(part 1 of 2)
# Autodesk Inventor assembly: testframe
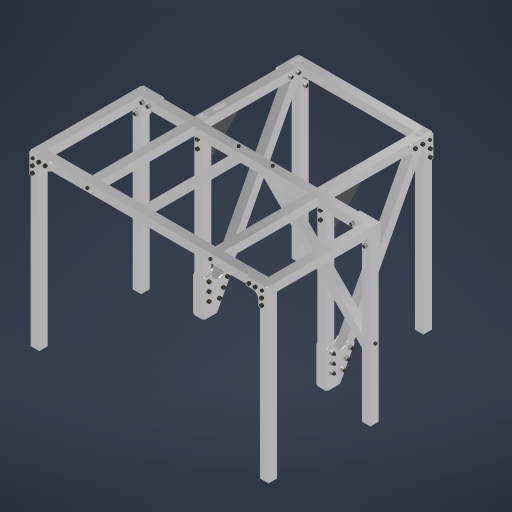
[picture p0: Inventor's stored thumbnail of the model, 512x512]
Saved by Autodesk Inventor 2024.2 (Build 282272000, 272)
## iProperties
Created: 2024-07-23
Part Number: testframe
Document SubType Name: Assembly
Designer: bryan
Mass: 9363.54 g
Surface Area: 20423.1 cm^2
Volume: 3333.5 cm^3
Density: 2.80893 g/cm^3
Author: bryan
## Documents named in this file (28)
- C:\Users\bobsb\OneDrive\Documents\GitHub\1622-2024-Summer-CAD-A-Thon\Structure\STRU_000_StructureAssembly.iam
- C:\Users\bobsb\OneDrive\Documents\GitHub\1622-2024-Summer-CAD-A-Thon\Structure\STRU_001_BilletBlock.ipt
- C:\Users\bobsb\OneDrive\Documents\GitHub\1622-2024-Summer-CAD-A-Thon\Structure\STRU_002_BilletPole_20.56in_Angled.ipt
- C:\Users\bobsb\OneDrive\Documents\GitHub\1622-2024-Summer-CAD-A-Thon\Structure\STRU_003_BilletPole_28in_Angled.ipt
- C:\Users\bobsb\OneDrive\Documents\GitHub\1622-2024-Summer-CAD-A-Thon\Structure\STRU_004_DoubleBillet_90_2.25in.ipt
- C:\Users\bobsb\OneDrive\Documents\GitHub\1622-2024-Summer-CAD-A-Thon\Structure\STRU_007_BilletPole_11in.ipt
- C:\Users\bobsb\OneDrive\Documents\GitHub\1622-2024-Summer-CAD-A-Thon\Structure\STRU_003_BilletPole_28in_Angled_Unique.ipt
- C:\Users\bobsb\OneDrive\Documents\GitHub\1622-2024-Summer-CAD-A-Thon\COTS Library\Fasteners\Bolts\Socket-Head\10-32\COTS_90044A120_Black-Oxide Alloy Steel Socket Head Screw.ipt
- C:\Users\bobsb\OneDrive\Documents\GitHub\1622-2024-Summer-CAD-A-Thon\COTS Library\Fasteners\Bolts\Socket-Head\0.25-20\COTS_90044A123_Black-Oxide Alloy Steel Socket Head Screw.ipt
- C:\Users\bobsb\OneDrive\Documents\GitHub\1622-2024-Summer-CAD-A-Thon\COTS Library\Fasteners\Nuts\COTS_95615A120_Medium-Strength Steel Nylon-Insert Locknut.ipt
- C:\Users\bobsb\OneDrive\Documents\GitHub\1622-2024-Summer-CAD-A-Thon\Structure\STRU_009_FrameBracket_90.ipt
- C:\Users\bobsb\OneDrive\Documents\GitHub\1622-2024-Summer-CAD-A-Thon\Structure\STRU_006_BilletPole_SwerveOffset.ipt
- C:\Users\bobsb\OneDrive\Documents\GitHub\1622-2024-Summer-CAD-A-Thon\Structure\STRU_010_BilletCrossbar_Angled.ipt
- C:\Users\bobsb\OneDrive\Documents\GitHub\1622-2024-Summer-CAD-A-Thon\Structure\STRU_011_BilletWedge.ipt
- C:\Users\bobsb\OneDrive\Documents\GitHub\1622-2024-Summer-CAD-A-Thon\COTS Library\Fasteners\Bolts\Socket-Head\10-32\COTS_90044A119_Black-Oxide Alloy Steel Socket Head Screw.ipt
- C:\Users\bobsb\OneDrive\Documents\GitHub\1622-2024-Summer-CAD-A-Thon\Structure\STRU_012_BilletPoleMiddle.ipt
- C:\Users\bobsb\OneDrive\Documents\GitHub\1622-2024-Summer-CAD-A-Thon\Structure\STRU_013_BilletCrossbar2_Angled.ipt
- C:\Users\bobsb\OneDrive\Documents\GitHub\1622-2024-Summer-CAD-A-Thon\Structure\STRU_012_BilletPoleMiddle_Unique.ipt
- C:\Users\bobsb\OneDrive\Documents\GitHub\1622-2024-Summer-CAD-A-Thon\Structure\STRU_014_BilletPole_9in_Angled.ipt
- C:\Users\bobsb\OneDrive\Documents\GitHub\1622-2024-Summer-CAD-A-Thon\Structure\STRU_015_BilletPole_9in.ipt
- C:\Users\bobsb\OneDrive\Documents\GitHub\1622-2024-Summer-CAD-A-Thon\Structure\STRU_016_FrameBracket2_90.ipt
- C:\Users\bobsb\OneDrive\Documents\GitHub\1622-2024-Summer-CAD-A-Thon\Structure\STRU_017_AngleBracket_90_Plastic.ipt
- C:\Users\bobsb\OneDrive\Documents\GitHub\1622-2024-Summer-CAD-A-Thon\Structure\STRU_018_AngleBracket_62.ipt
- C:\Users\bobsb\OneDrive\Documents\GitHub\1622-2024-Summer-CAD-A-Thon\COTS Library\Fasteners\Bolts\Socket-Head\0.25-20\COTS_91251A539_Black-Oxide Alloy Steel Socket Head Screw (1).ipt
- C:\Users\bobsb\OneDrive\Documents\GitHub\1622-2024-Summer-CAD-A-Thon\COTS Library\Fasteners\Bolts\Socket-Head\0.25-20\COTS_90044A124_Black-Oxide Alloy Steel Socket Head Screw.ipt
- C:\Users\bobsb\OneDrive\Documents\GitHub\1622-2024-Summer-CAD-A-Thon\COTS Library\Fasteners\Nuts\COTS_95462A029_Medium-Strength Steel Hex Nut (2).ipt
- C:\Users\bobsb\OneDrive\Documents\GitHub\1622-2024-Summer-CAD-A-Thon\Structure\STRU_019_RubberWasher.ipt
- C:\Users\bobsb\OneDrive\Documents\GitHub\1622-2024-Summer-CAD-A-Thon\Structure\STRU_000_StructureAssembly\AIP\FEA\err5tqxb5.fres
## Components (169 placed, 26 different names)
1. STRU_001_BilletBlock:2 — Mate:16, Mate:17, Flush:2
2. STRU_002_BilletPole_20.56in_Angled:1 — Mate:1, Mate:4, Mate:5, Mate:41, Mate:53, Mate:54, Flush:10, Mate:91, Mate:92, Mate:127, Mate:147, Mate:148, Mate:209, Mate:211, Mate:212, Mate:213, Mate:411
3. STRU_004_DoubleBillet_90_2.25in:1 — Mate:1, Mate:4, Mate:5, Mate:34, Mate:56, Mate:58, Mate:125, Mate:126
4. STRU_002_BilletPole_20.56in_Angled:2 — Mate:13, Mate:14, Mate:15, Mate:16, Mate:17, Flush:2, Mate:40, Mate:85, Mate:86, Mate:123, Mate:124, Mate:145, Mate:146, Mate:200, Mate:201, Mate:218, Mate:219, Mate:415
5. STRU_004_DoubleBillet_90_2.25in:2 — Mate:13, Mate:14, Mate:15, Mate:36, Mate:57, Mate:100, Mate:121, Mate:122
6. STRU_001_BilletBlock:3 — Mate:185, Mate:186, Flush:26
7. STRU_001_BilletBlock:4 — Mate:180, Mate:181, Flush:25
8. STRU_003_BilletPole_28in_Angled:2 — Mate:47, Flush:8, Flush:9, Mate:55, Mate:74, Mate:79, Mate:80, Mate:87, Mate:88, Mate:97, Mate:118, Mate:130, Mate:140, Mate:153, Mate:154, Mate:155, Mate:156, Mate:157, Mate:158, Mate:161, Mate:163, Mate:168, Mate:173, Flush:24, Mate:176, Mate:178, Mate:182
9. STRU_004_DoubleBillet_90_2.25in:3 — Mate:35, Mate:128, Mate:129, Mate:184
10. STRU_004_DoubleBillet_90_2.25in:4 — Mate:37, Mate:119, Mate:120, Mate:179
11. STRU_001_BilletBlock:5 — Mate:34, Mate:41, Mate:50, Mate:51
12. STRU_001_BilletBlock:6 — Mate:35, Mate:48, Mate:49
13. STRU_001_BilletBlock:7 — Mate:37, Mate:45, Mate:46
14. STRU_001_BilletBlock:8 — Mate:36, Mate:40, Mate:42, Mate:43
15. STRU_007_BilletPole_11in:1 — Mate:48, Mate:49, Flush:9, Mate:50, Mate:51, Mate:55, Mate:59
16. STRU_007_BilletPole_11in:2 — Mate:42, Mate:43, Mate:45, Mate:46, Mate:47, Flush:8, Mate:124
17. STRU_001_BilletBlock:9 — Mate:53, Mate:54, Flush:10
18. STRU_003_BilletPole_28in_Angled_Unique:1 — Mate:56, Mate:57, Mate:58, Mate:59, Mate:83, Mate:84, Mate:93, Mate:94, Mate:98, Mate:149, Mate:150, Mate:151, Mate:152, Mate:159, Mate:160, Mate:164, Mate:165, Flush:27, Mate:203, Mate:205, Mate:206, Mate:208, Mate:214, Mate:215, Mate:216, Mate:217, Flush:28, Mate:221, Flush:29, Mate:223, Mate:261, Mate:262, Mate:408, Mate:412
19. STRU_001_BilletBlock:10 — Mate:74, Mate:157, Mate:172
20. COTS_90044A120_Black-Oxide Alloy Steel Socket Head Screw:1 — Mate:142, Mate:193
21. COTS_90044A123_Black-Oxide Alloy Steel Socket Head Screw:2 — Mate:80, Mate:102, Mate:141, Flush:21
22. COTS_90044A123_Black-Oxide Alloy Steel Socket Head Screw:3 — Mate:103, Flush:22, Flush:23, Mate:191
23. COTS_90044A123_Black-Oxide Alloy Steel Socket Head Screw:4 — Mate:79, Mate:101, Flush:21, Flush:22
24. COTS_90044A123_Black-Oxide Alloy Steel Socket Head Screw:5 — Mate:104, Flush:23, Mate:192
25. COTS_90044A123_Black-Oxide Alloy Steel Socket Head Screw:6 — Mate:84, Mate:108, Flush:12
26. COTS_90044A123_Black-Oxide Alloy Steel Socket Head Screw:7 — Mate:85, Mate:106, Mate:134, Flush:12, Flush:13, Flush:14
27. COTS_90044A123_Black-Oxide Alloy Steel Socket Head Screw:8 — Mate:83, Mate:107, Flush:13
28. COTS_90044A123_Black-Oxide Alloy Steel Socket Head Screw:9 — Mate:86, Mate:105, Flush:14
29. COTS_90044A123_Black-Oxide Alloy Steel Socket Head Screw:10 — Mate:112, Flush:18, Mate:188
30. COTS_90044A123_Black-Oxide Alloy Steel Socket Head Screw:11 — Mate:111, Mate:139, Flush:18, Flush:19, Flush:20, Mate:187
31. COTS_90044A123_Black-Oxide Alloy Steel Socket Head Screw:12 — Mate:88, Mate:110, Flush:20
32. COTS_90044A123_Black-Oxide Alloy Steel Socket Head Screw:13 — Mate:87, Mate:109, Flush:19
33. COTS_90044A123_Black-Oxide Alloy Steel Socket Head Screw:14 — Mate:93, Mate:115, Flush:16
34. COTS_90044A123_Black-Oxide Alloy Steel Socket Head Screw:15 — Mate:92, Mate:114, Flush:17
35. COTS_90044A123_Black-Oxide Alloy Steel Socket Head Screw:16 — Mate:91, Mate:113, Mate:136, Flush:15, Flush:17
36. COTS_90044A123_Black-Oxide Alloy Steel Socket Head Screw:17 — Mate:94, Mate:116, Flush:15, Flush:16
37. COTS_90044A120_Black-Oxide Alloy Steel Socket Head Screw:3 — Mate:140, Mate:158
38. COTS_90044A120_Black-Oxide Alloy Steel Socket Head Screw:5 — Mate:97, Mate:138
39. COTS_90044A120_Black-Oxide Alloy Steel Socket Head Screw:6 — Mate:100, Mate:135
40. COTS_90044A120_Black-Oxide Alloy Steel Socket Head Screw:7 — Mate:98, Mate:137
41. COTS_95615A120_Medium-Strength Steel Nylon-Insert Locknut:1 — Mate:102, Mate:154
42. COTS_95615A120_Medium-Strength Steel Nylon-Insert Locknut:2 — Mate:101, Mate:153
43. COTS_95615A120_Medium-Strength Steel Nylon-Insert Locknut:3 — Mate:103, Mate:194
44. COTS_95615A120_Medium-Strength Steel Nylon-Insert Locknut:4 — Mate:104, Mate:195
45. COTS_95615A120_Medium-Strength Steel Nylon-Insert Locknut:5 — Mate:107, Mate:152
46. COTS_95615A120_Medium-Strength Steel Nylon-Insert Locknut:6 — Mate:108, Mate:151
47. COTS_95615A120_Medium-Strength Steel Nylon-Insert Locknut:7 — Mate:105, Mate:145
48. COTS_95615A120_Medium-Strength Steel Nylon-Insert Locknut:8 — Mate:106, Mate:146
49. COTS_95615A120_Medium-Strength Steel Nylon-Insert Locknut:9 — Mate:109, Mate:155
50. COTS_95615A120_Medium-Strength Steel Nylon-Insert Locknut:10 — Mate:110, Mate:156
51. COTS_95615A120_Medium-Strength Steel Nylon-Insert Locknut:11 — Mate:111, Mate:189
52. COTS_95615A120_Medium-Strength Steel Nylon-Insert Locknut:12 — Mate:112, Mate:190
53. COTS_95615A120_Medium-Strength Steel Nylon-Insert Locknut:13 — Mate:114, Mate:147
54. COTS_95615A120_Medium-Strength Steel Nylon-Insert Locknut:14 — Mate:113, Mate:148
55. COTS_95615A120_Medium-Strength Steel Nylon-Insert Locknut:15 — Mate:115, Mate:149
56. COTS_95615A120_Medium-Strength Steel Nylon-Insert Locknut:16 — Mate:116, Mate:150
57. STRU_009_FrameBracket_90:1 — Mate:118, Mate:119, Mate:120, Mate:141, Mate:142, Mate:177, Mate:191, Mate:192, Mate:193
58. STRU_009_FrameBracket_90:2 — Mate:125, Mate:126, Mate:127, Mate:136, Mate:137
59. STRU_009_FrameBracket_90:3 — Mate:121, Mate:122, Mate:123, Mate:134, Mate:135
60. STRU_009_FrameBracket_90:4 — Mate:128, Mate:129, Mate:130, Mate:138, Mate:139, Mate:183, Mate:187, Mate:188
61. STRU_001_BilletBlock:11 — Mate:159, Mate:165, Mate:171
62. STRU_001_BilletBlock:12 — Mate:160, Mate:164, Mate:174
63. STRU_001_BilletBlock:13 — Mate:161, Mate:162, Mate:163, Mate:175
64. COTS_90044A120_Black-Oxide Alloy Steel Socket Head Screw:10 — Mate:162, Mate:168
65. STRU_007_BilletPole_11in:3 — Mate:171, Mate:172, Mate:173, Flush:27
66. STRU_007_BilletPole_11in:4 — Mate:174, Mate:175, Flush:24, Mate:176
67. STRU_006_BilletPole_SwerveOffset:1 — Mate:177, Mate:178, Mate:179, Mate:180, Mate:181, Flush:25, Mate:194, Mate:195
68. STRU_006_BilletPole_SwerveOffset:2 — Mate:182, Mate:183, Mate:184, Mate:185, Mate:186, Flush:26, Mate:189, Mate:190
69. STRU_011_BilletWedge:1 — Mate:200, Mate:201, Mate:414
70. STRU_011_BilletWedge:3 — Mate:203, Mate:205, Mate:413
71. STRU_011_BilletWedge:4 — Mate:206, Mate:208, Mate:409
72. STRU_011_BilletWedge:5 — Mate:209, Mate:211, Mate:410
73. COTS_90044A119_Black-Oxide Alloy Steel Socket Head Screw:1 — Mate:212, Mate:213
74. COTS_90044A119_Black-Oxide Alloy Steel Socket Head Screw:2 — Mate:214, Mate:215
75. COTS_90044A119_Black-Oxide Alloy Steel Socket Head Screw:3 — Mate:216, Mate:217
76. COTS_90044A119_Black-Oxide Alloy Steel Socket Head Screw:4 — Mate:218, Mate:219
77. STRU_012_BilletPoleMiddle:6 — Flush:28, Mate:221, Mate:228, Mate:229, Flush:30, Flush:43, Mate:251, Mate:255, Flush:49, Mate:261, Mate:263, Mate:318, Mate:324, Mate:331, Mate:389, Mate:390, Mate:418, Mate:419
78. STRU_012_BilletPoleMiddle:5 — Flush:29, Mate:223, Mate:230, Mate:231, Flush:31, Flush:39, Mate:233, Mate:234, Mate:249, Mate:253, Flush:48, Mate:262, Mate:264, Mate:319, Mate:321, Mate:328, Mate:391, Mate:392, Mate:416, Mate:417
79. STRU_001_BilletBlock:14 — Mate:228, Mate:229, Flush:30
80. STRU_001_BilletBlock:15 — Mate:230, Mate:231, Flush:31
81. STRU_013_BilletCrossbar2_Angled:1 — Flush:39, Mate:233, Mate:234, Mate:252, Mate:273, Flush:56, Flush:57, Mate:287, Mate:322, Mate:323, Mate:327, Mate:329
82. STRU_013_BilletCrossbar2_Angled:3 — Flush:43, Mate:254, Mate:274, Flush:58, Mate:308, Mate:325, Mate:326, Mate:330, Mate:332
83. STRU_001_BilletBlock:16 — Mate:267, Mate:268, Flush:54
84. STRU_001_BilletBlock:17 — Mate:269, Mate:270, Flush:55
85. COTS_90044A120_Black-Oxide Alloy Steel Socket Head Screw:11 — Mate:249, Mate:264
86. COTS_90044A120_Black-Oxide Alloy Steel Socket Head Screw:12 — Mate:251, Mate:263
87. STRU_014_BilletPole_9in_Angled:1 — Mate:254, Mate:255, Flush:49, Mate:311, Mate:317, Mate:333, Mate:334, Mate:335, Mate:336
88. STRU_014_BilletPole_9in_Angled:2 — Mate:252, Mate:253, Flush:48, Mate:291, Mate:320, Mate:337, Mate:338, Mate:339, Mate:340
89. STRU_015_BilletPole_9in:1 — Mate:257, Mate:258, Mate:259, Mate:260, Flush:52, Flush:53, Flush:57
90. STRU_001_BilletBlock:18 — Mate:259, Mate:260, Flush:52, Mate:266, Mate:271, Mate:275
91. STRU_001_BilletBlock:19 — Mate:257, Mate:258, Flush:53, Mate:265, Mate:272, Mate:276
92. STRU_012_BilletPoleMiddle_Unique:1 — Mate:265, Mate:267, Mate:268, Flush:54, Mate:272, Mate:274, Flush:58, Mate:277, Mate:278, Mate:279, Mate:304, Mate:316
93. STRU_012_BilletPoleMiddle_Unique:2 — Mate:266, Mate:269, Mate:270, Flush:55, Mate:271, Mate:273, Flush:56, Mate:281, Mate:282, Mate:283, Mate:295, Mate:299
94. COTS_90044A120_Black-Oxide Alloy Steel Socket Head Screw:13 — Mate:275, Mate:284
95. COTS_90044A120_Black-Oxide Alloy Steel Socket Head Screw:14 — Mate:276, Mate:280
96. STRU_016_FrameBracket2_90:1 — Mate:277, Mate:278, Mate:279, Mate:280, Mate:302, Mate:303, Mate:306, Mate:307, Mate:310, Mate:312, Mate:314, Mate:315
97. STRU_016_FrameBracket2_90:2 — Mate:281, Mate:282, Mate:283, Mate:284, Mate:286, Mate:288, Mate:290, Mate:292, Mate:294, Mate:296, Mate:298, Mate:300
98. COTS_90044A123_Black-Oxide Alloy Steel Socket Head Screw:18 — Mate:286, Mate:288
99. COTS_95615A120_Medium-Strength Steel Nylon-Insert Locknut:17 — Mate:287
100. COTS_90044A123_Black-Oxide Alloy Steel Socket Head Screw:19 — Mate:290, Mate:292
101. COTS_95615A120_Medium-Strength Steel Nylon-Insert Locknut:18 — Mate:291
102. COTS_90044A123_Black-Oxide Alloy Steel Socket Head Screw:20 — Mate:294, Mate:296
103. COTS_95615A120_Medium-Strength Steel Nylon-Insert Locknut:19 — Mate:295
104. COTS_90044A123_Black-Oxide Alloy Steel Socket Head Screw:21 — Mate:298, Mate:300
105. COTS_95615A120_Medium-Strength Steel Nylon-Insert Locknut:20 — Mate:299
106. COTS_90044A123_Black-Oxide Alloy Steel Socket Head Screw:22 — Mate:302, Mate:303
107. COTS_95615A120_Medium-Strength Steel Nylon-Insert Locknut:21 — Mate:304
108. COTS_90044A123_Black-Oxide Alloy Steel Socket Head Screw:23 — Mate:306, Mate:307
109. COTS_95615A120_Medium-Strength Steel Nylon-Insert Locknut:22 — Mate:308
110. COTS_90044A123_Black-Oxide Alloy Steel Socket Head Screw:24 — Mate:310, Mate:312
111. COTS_95615A120_Medium-Strength Steel Nylon-Insert Locknut:23 — Mate:311
112. COTS_90044A123_Black-Oxide Alloy Steel Socket Head Screw:25 — Mate:314, Mate:315
113. COTS_95615A120_Medium-Strength Steel Nylon-Insert Locknut:24 — Mate:316
114. STRU_017_AngleBracket_90_Plastic:1 — Mate:317, Mate:318, Mate:453, Mate:454, Mate:458, Mate:462, Mate:463, Mate:467
115. STRU_017_AngleBracket_90_Plastic:2 — Mate:319, Mate:320, Mate:434, Mate:435, Mate:440, Mate:444, Mate:445, Mate:449
116. STRU_018_AngleBracket_62:1 — Mate:327, Mate:328, Mate:329, Mate:393, Mate:394, Mate:395, Mate:396, Mate:397, Mate:398, Mate:399, Mate:400, Mate:401, Mate:402, Mate:403, Mate:404
117. STRU_018_AngleBracket_62:2 — Mate:330, Mate:331, Mate:332, Mate:359, Mate:360, Mate:361, Mate:362, Mate:363, Mate:364, Mate:383, Mate:384, Mate:385, Mate:386, Mate:387, Mate:388
118. STRU_018_AngleBracket_62:3 — Mate:321, Mate:322, Mate:323, Mate:426, Mate:427, Mate:428, Mate:429, Mate:430, Mate:431
119. STRU_018_AngleBracket_62:4 — Mate:324, Mate:325, Mate:326, Mate:377, Mate:378, Mate:379, Mate:380, Mate:381, Mate:382
120. COTS_91251A539_Black-Oxide Alloy Steel Socket Head Screw (1):1 — Mate:337, Mate:340, Mate:439
121. COTS_91251A539_Black-Oxide Alloy Steel Socket Head Screw (1):2 — Mate:338, Mate:339, Mate:432, Mate:433
122. COTS_91251A539_Black-Oxide Alloy Steel Socket Head Screw (1):4 — Mate:333, Mate:334, Mate:457
123. COTS_91251A539_Black-Oxide Alloy Steel Socket Head Screw (1):5 — Mate:335, Mate:336, Mate:452
124. COTS_95615A120_Medium-Strength Steel Nylon-Insert Locknut:25 — Mate:373, Mate:385
125. COTS_95615A120_Medium-Strength Steel Nylon-Insert Locknut:26 — Mate:372, Mate:384
126. COTS_95615A120_Medium-Strength Steel Nylon-Insert Locknut:27 — Mate:371, Mate:383
127. COTS_95615A120_Medium-Strength Steel Nylon-Insert Locknut:28 — Mate:376, Mate:388
128. COTS_95615A120_Medium-Strength Steel Nylon-Insert Locknut:29 — Mate:375, Mate:387
129. COTS_95615A120_Medium-Strength Steel Nylon-Insert Locknut:30 — Mate:374, Mate:386
130. COTS_90044A123_Black-Oxide Alloy Steel Socket Head Screw:27 — Mate:390, Mate:419, Mate:461
131. COTS_90044A123_Black-Oxide Alloy Steel Socket Head Screw:28 — Mate:389, Mate:418, Mate:466
132. COTS_90044A123_Black-Oxide Alloy Steel Socket Head Screw:29 — Mate:392, Mate:417, Mate:448
133. COTS_90044A123_Black-Oxide Alloy Steel Socket Head Screw:30 — Mate:391, Mate:416, Mate:442, Mate:443
134. COTS_90044A124_Black-Oxide Alloy Steel Socket Head Screw:1 — Mate:359, Mate:371, Mate:382
135. COTS_90044A124_Black-Oxide Alloy Steel Socket Head Screw:2 — Mate:361, Mate:373, Mate:378
136. COTS_90044A124_Black-Oxide Alloy Steel Socket Head Screw:3 — Mate:360, Mate:372, Mate:381
137. COTS_90044A124_Black-Oxide Alloy Steel Socket Head Screw:4 — Mate:393, Mate:399, Mate:421
138. COTS_90044A124_Black-Oxide Alloy Steel Socket Head Screw:5 — Mate:394, Mate:401, Mate:422
139. COTS_90044A124_Black-Oxide Alloy Steel Socket Head Screw:6 — Mate:395, Mate:400, Mate:423
140. COTS_90044A124_Black-Oxide Alloy Steel Socket Head Screw:7 — Mate:362, Mate:374, Mate:379
141. COTS_90044A124_Black-Oxide Alloy Steel Socket Head Screw:8 — Mate:363, Mate:375, Mate:380
142. COTS_90044A124_Black-Oxide Alloy Steel Socket Head Screw:9 — Mate:364, Mate:376, Mate:377
143. COTS_90044A124_Black-Oxide Alloy Steel Socket Head Screw:10 — Mate:396, Mate:404, Mate:425
144. COTS_90044A124_Black-Oxide Alloy Steel Socket Head Screw:11 — Mate:397, Mate:403, Mate:424
145. COTS_90044A124_Black-Oxide Alloy Steel Socket Head Screw:12 — Mate:398, Mate:402, Mate:420
146. STRU_010_BilletCrossbar_Angled:2 — Mate:408, Mate:409, Mate:410, Mate:411
147. STRU_010_BilletCrossbar_Angled:3 — Mate:412, Mate:413, Mate:414, Mate:415
148. COTS_95615A120_Medium-Strength Steel Nylon-Insert Locknut:31 — Mate:423, Mate:430
149. COTS_95615A120_Medium-Strength Steel Nylon-Insert Locknut:32 — Mate:421, Mate:426
150. COTS_95615A120_Medium-Strength Steel Nylon-Insert Locknut:33 — Mate:425, Mate:429
151. COTS_95615A120_Medium-Strength Steel Nylon-Insert Locknut:34 — Mate:420, Mate:427
152. COTS_95615A120_Medium-Strength Steel Nylon-Insert Locknut:35 — Mate:422, Mate:431
153. COTS_95615A120_Medium-Strength Steel Nylon-Insert Locknut:36 — Mate:424, Mate:428
154. COTS_95462A029_Medium-Strength Steel Hex Nut (2):1 — Mate:432, Mate:436
155. STRU_019_RubberWasher:1 — Mate:433, Mate:434, Mate:435, Mate:436, Flush:59
156. COTS_95462A029_Medium-Strength Steel Hex Nut (2):2 — Mate:438, Mate:439
157. STRU_019_RubberWasher:2 — Mate:438, Flush:59, Mate:440
158. COTS_95462A029_Medium-Strength Steel Hex Nut (2):3 — Mate:442
159. STRU_019_RubberWasher:3 — Mate:443, Mate:444, Mate:445, Flush:60
160. COTS_95462A029_Medium-Strength Steel Hex Nut (2):4 — Mate:447, Mate:448
161. STRU_019_RubberWasher:4 — Mate:447, Mate:449, Flush:60
162. COTS_95462A029_Medium-Strength Steel Hex Nut (2):5 — Mate:452
163. STRU_019_RubberWasher:5 — Mate:453, Mate:454, Flush:61
164. COTS_95462A029_Medium-Strength Steel Hex Nut (2):6 — Mate:457
165. STRU_019_RubberWasher:6 — Mate:458, Flush:61
166. COTS_95462A029_Medium-Strength Steel Hex Nut (2):7 — Mate:461
167. STRU_019_RubberWasher:7 — Mate:462, Mate:463, Flush:62
168. COTS_95462A029_Medium-Strength Steel Hex Nut (2):8 — Mate:466
169. STRU_019_RubberWasher:8 — Mate:467, Flush:62
## Relationships (390: Mate 351, Flush 39)
- Mate:1: STRU_002_BilletPole_20.56in_Angled:1 ↔ STRU_004_DoubleBillet_90_2.25in:1
- Mate:4: STRU_002_BilletPole_20.56in_Angled:1 ↔ STRU_004_DoubleBillet_90_2.25in:1
- Mate:5: STRU_002_BilletPole_20.56in_Angled:1 ↔ STRU_004_DoubleBillet_90_2.25in:1
- Mate:13: STRU_002_BilletPole_20.56in_Angled:2 ↔ STRU_004_DoubleBillet_90_2.25in:2
- Mate:14: STRU_002_BilletPole_20.56in_Angled:2 ↔ STRU_004_DoubleBillet_90_2.25in:2
- Mate:15: STRU_002_BilletPole_20.56in_Angled:2 ↔ STRU_004_DoubleBillet_90_2.25in:2
- Mate:16: STRU_001_BilletBlock:2 ↔ STRU_002_BilletPole_20.56in_Angled:2
- Mate:17: STRU_001_BilletBlock:2 ↔ STRU_002_BilletPole_20.56in_Angled:2
- Flush:2: STRU_001_BilletBlock:2 ↔ STRU_002_BilletPole_20.56in_Angled:2
- [Mate]: STRU_003_BilletPole_28in_Angled:2 ↔ STRU_004_DoubleBillet_90_2.25in:3
- [Mate]: STRU_003_BilletPole_28in_Angled:2 ↔ STRU_004_DoubleBillet_90_2.25in:3
- [Mate]: STRU_003_BilletPole_28in_Angled:2 ↔ STRU_004_DoubleBillet_90_2.25in:3
- [Mate]: STRU_003_BilletPole_28in_Angled:2 ↔ STRU_004_DoubleBillet_90_2.25in:4
- [Mate]: STRU_003_BilletPole_28in_Angled:2 ↔ STRU_004_DoubleBillet_90_2.25in:4
- [Mate]: STRU_003_BilletPole_28in_Angled:2 ↔ STRU_004_DoubleBillet_90_2.25in:4
- Mate:34: STRU_004_DoubleBillet_90_2.25in:1 ↔ STRU_001_BilletBlock:5
- Mate:35: STRU_004_DoubleBillet_90_2.25in:3 ↔ STRU_001_BilletBlock:6
- Mate:36: STRU_004_DoubleBillet_90_2.25in:2 ↔ STRU_001_BilletBlock:8
- Mate:37: STRU_004_DoubleBillet_90_2.25in:4 ↔ STRU_001_BilletBlock:7
- Mate:40: STRU_002_BilletPole_20.56in_Angled:2 ↔ STRU_001_BilletBlock:8
- Mate:41: STRU_002_BilletPole_20.56in_Angled:1 ↔ STRU_001_BilletBlock:5
- Mate:42: STRU_001_BilletBlock:8 ↔ STRU_007_BilletPole_11in:2
- Mate:43: STRU_001_BilletBlock:8 ↔ STRU_007_BilletPole_11in:2
- Mate:45: STRU_001_BilletBlock:7 ↔ STRU_007_BilletPole_11in:2
- Mate:46: STRU_001_BilletBlock:7 ↔ STRU_007_BilletPole_11in:2
- Mate:47: STRU_003_BilletPole_28in_Angled:2 ↔ STRU_007_BilletPole_11in:2
- Flush:8: STRU_003_BilletPole_28in_Angled:2 ↔ STRU_007_BilletPole_11in:2
- Mate:48: STRU_001_BilletBlock:6 ↔ STRU_007_BilletPole_11in:1
- Mate:49: STRU_001_BilletBlock:6 ↔ STRU_007_BilletPole_11in:1
- Flush:9: STRU_003_BilletPole_28in_Angled:2 ↔ STRU_007_BilletPole_11in:1
- Mate:50: STRU_001_BilletBlock:5 ↔ STRU_007_BilletPole_11in:1
- Mate:51: STRU_001_BilletBlock:5 ↔ STRU_007_BilletPole_11in:1
- Mate:53: STRU_002_BilletPole_20.56in_Angled:1 ↔ STRU_001_BilletBlock:9
- Mate:54: STRU_002_BilletPole_20.56in_Angled:1 ↔ STRU_001_BilletBlock:9
- Flush:10: STRU_002_BilletPole_20.56in_Angled:1 ↔ STRU_001_BilletBlock:9
- Mate:55: STRU_003_BilletPole_28in_Angled:2 ↔ STRU_007_BilletPole_11in:1
- Mate:56: STRU_004_DoubleBillet_90_2.25in:1 ↔ STRU_003_BilletPole_28in_Angled_Unique:1
- Mate:57: STRU_004_DoubleBillet_90_2.25in:2 ↔ STRU_003_BilletPole_28in_Angled_Unique:1
- Mate:58: STRU_004_DoubleBillet_90_2.25in:1 ↔ STRU_003_BilletPole_28in_Angled_Unique:1
- Mate:59: STRU_007_BilletPole_11in:1 ↔ STRU_003_BilletPole_28in_Angled_Unique:1
- Mate:74: STRU_003_BilletPole_28in_Angled:2 ↔ STRU_001_BilletBlock:10
- Mate:79: STRU_003_BilletPole_28in_Angled:2 ↔ COTS_90044A123_Black-Oxide Alloy Steel Socket Head Screw:4
- Mate:80: STRU_003_BilletPole_28in_Angled:2 ↔ COTS_90044A123_Black-Oxide Alloy Steel Socket Head Screw:2
- Mate:83: STRU_003_BilletPole_28in_Angled_Unique:1 ↔ COTS_90044A123_Black-Oxide Alloy Steel Socket Head Screw:8
- Mate:84: STRU_003_BilletPole_28in_Angled_Unique:1 ↔ COTS_90044A123_Black-Oxide Alloy Steel Socket Head Screw:6
- Mate:85: STRU_002_BilletPole_20.56in_Angled:2 ↔ COTS_90044A123_Black-Oxide Alloy Steel Socket Head Screw:7
- Mate:86: STRU_002_BilletPole_20.56in_Angled:2 ↔ COTS_90044A123_Black-Oxide Alloy Steel Socket Head Screw:9
- Mate:87: STRU_003_BilletPole_28in_Angled:2 ↔ COTS_90044A123_Black-Oxide Alloy Steel Socket Head Screw:13
- Mate:88: STRU_003_BilletPole_28in_Angled:2 ↔ COTS_90044A123_Black-Oxide Alloy Steel Socket Head Screw:12
- Mate:91: STRU_002_BilletPole_20.56in_Angled:1 ↔ COTS_90044A123_Black-Oxide Alloy Steel Socket Head Screw:16
- Mate:92: STRU_002_BilletPole_20.56in_Angled:1 ↔ COTS_90044A123_Black-Oxide Alloy Steel Socket Head Screw:15
- Mate:93: STRU_003_BilletPole_28in_Angled_Unique:1 ↔ COTS_90044A123_Black-Oxide Alloy Steel Socket Head Screw:14
- Mate:94: STRU_003_BilletPole_28in_Angled_Unique:1 ↔ COTS_90044A123_Black-Oxide Alloy Steel Socket Head Screw:17
- Mate:97: STRU_003_BilletPole_28in_Angled:2 ↔ COTS_90044A120_Black-Oxide Alloy Steel Socket Head Screw:5
- Mate:98: STRU_003_BilletPole_28in_Angled_Unique:1 ↔ COTS_90044A120_Black-Oxide Alloy Steel Socket Head Screw:7
- Mate:100: STRU_004_DoubleBillet_90_2.25in:2 ↔ COTS_90044A120_Black-Oxide Alloy Steel Socket Head Screw:6
- Mate:101: COTS_90044A123_Black-Oxide Alloy Steel Socket Head Screw:4 ↔ COTS_95615A120_Medium-Strength Steel Nylon-Insert Locknut:2
- Mate:102: COTS_90044A123_Black-Oxide Alloy Steel Socket Head Screw:2 ↔ COTS_95615A120_Medium-Strength Steel Nylon-Insert Locknut:1
- Mate:103: COTS_90044A123_Black-Oxide Alloy Steel Socket Head Screw:3 ↔ COTS_95615A120_Medium-Strength Steel Nylon-Insert Locknut:3
- Mate:104: COTS_90044A123_Black-Oxide Alloy Steel Socket Head Screw:5 ↔ COTS_95615A120_Medium-Strength Steel Nylon-Insert Locknut:4
- Mate:105: COTS_90044A123_Black-Oxide Alloy Steel Socket Head Screw:9 ↔ COTS_95615A120_Medium-Strength Steel Nylon-Insert Locknut:7
- Mate:106: COTS_90044A123_Black-Oxide Alloy Steel Socket Head Screw:7 ↔ COTS_95615A120_Medium-Strength Steel Nylon-Insert Locknut:8
- Mate:107: COTS_90044A123_Black-Oxide Alloy Steel Socket Head Screw:8 ↔ COTS_95615A120_Medium-Strength Steel Nylon-Insert Locknut:5
- Mate:108: COTS_90044A123_Black-Oxide Alloy Steel Socket Head Screw:6 ↔ COTS_95615A120_Medium-Strength Steel Nylon-Insert Locknut:6
- Mate:109: COTS_90044A123_Black-Oxide Alloy Steel Socket Head Screw:13 ↔ COTS_95615A120_Medium-Strength Steel Nylon-Insert Locknut:9
- Mate:110: COTS_90044A123_Black-Oxide Alloy Steel Socket Head Screw:12 ↔ COTS_95615A120_Medium-Strength Steel Nylon-Insert Locknut:10
- Mate:111: COTS_90044A123_Black-Oxide Alloy Steel Socket Head Screw:11 ↔ COTS_95615A120_Medium-Strength Steel Nylon-Insert Locknut:11
- Mate:112: COTS_90044A123_Black-Oxide Alloy Steel Socket Head Screw:10 ↔ COTS_95615A120_Medium-Strength Steel Nylon-Insert Locknut:12
- Mate:113: COTS_90044A123_Black-Oxide Alloy Steel Socket Head Screw:16 ↔ COTS_95615A120_Medium-Strength Steel Nylon-Insert Locknut:14
- Mate:114: COTS_90044A123_Black-Oxide Alloy Steel Socket Head Screw:15 ↔ COTS_95615A120_Medium-Strength Steel Nylon-Insert Locknut:13
- Mate:115: COTS_90044A123_Black-Oxide Alloy Steel Socket Head Screw:14 ↔ COTS_95615A120_Medium-Strength Steel Nylon-Insert Locknut:15
- Mate:116: COTS_90044A123_Black-Oxide Alloy Steel Socket Head Screw:17 ↔ COTS_95615A120_Medium-Strength Steel Nylon-Insert Locknut:16
- Mate:118: STRU_003_BilletPole_28in_Angled:2 ↔ STRU_009_FrameBracket_90:1
- Mate:119: STRU_004_DoubleBillet_90_2.25in:4 ↔ STRU_009_FrameBracket_90:1
- Mate:120: STRU_004_DoubleBillet_90_2.25in:4 ↔ STRU_009_FrameBracket_90:1
- Mate:121: STRU_004_DoubleBillet_90_2.25in:2 ↔ STRU_009_FrameBracket_90:3
- Mate:122: STRU_004_DoubleBillet_90_2.25in:2 ↔ STRU_009_FrameBracket_90:3
- Mate:123: STRU_002_BilletPole_20.56in_Angled:2 ↔ STRU_009_FrameBracket_90:3
- Mate:124: STRU_002_BilletPole_20.56in_Angled:2 ↔ STRU_007_BilletPole_11in:2
- Mate:125: STRU_004_DoubleBillet_90_2.25in:1 ↔ STRU_009_FrameBracket_90:2
- Mate:126: STRU_004_DoubleBillet_90_2.25in:1 ↔ STRU_009_FrameBracket_90:2
- Mate:127: STRU_002_BilletPole_20.56in_Angled:1 ↔ STRU_009_FrameBracket_90:2
- Mate:128: STRU_004_DoubleBillet_90_2.25in:3 ↔ STRU_009_FrameBracket_90:4
- Mate:129: STRU_004_DoubleBillet_90_2.25in:3 ↔ STRU_009_FrameBracket_90:4
- Mate:130: STRU_003_BilletPole_28in_Angled:2 ↔ STRU_009_FrameBracket_90:4
- Mate:134: COTS_90044A123_Black-Oxide Alloy Steel Socket Head Screw:7 ↔ STRU_009_FrameBracket_90:3
- Flush:12: COTS_90044A123_Black-Oxide Alloy Steel Socket Head Screw:6 ↔ COTS_90044A123_Black-Oxide Alloy Steel Socket Head Screw:7
- Mate:135: COTS_90044A120_Black-Oxide Alloy Steel Socket Head Screw:6 ↔ STRU_009_FrameBracket_90:3
- Flush:13: COTS_90044A123_Black-Oxide Alloy Steel Socket Head Screw:7 ↔ COTS_90044A123_Black-Oxide Alloy Steel Socket Head Screw:8
- Flush:14: COTS_90044A123_Black-Oxide Alloy Steel Socket Head Screw:7 ↔ COTS_90044A123_Black-Oxide Alloy Steel Socket Head Screw:9
- Mate:136: COTS_90044A123_Black-Oxide Alloy Steel Socket Head Screw:16 ↔ STRU_009_FrameBracket_90:2
- Mate:137: COTS_90044A120_Black-Oxide Alloy Steel Socket Head Screw:7 ↔ STRU_009_FrameBracket_90:2
- Flush:15: COTS_90044A123_Black-Oxide Alloy Steel Socket Head Screw:16 ↔ COTS_90044A123_Black-Oxide Alloy Steel Socket Head Screw:17
- Flush:16: COTS_90044A123_Black-Oxide Alloy Steel Socket Head Screw:14 ↔ COTS_90044A123_Black-Oxide Alloy Steel Socket Head Screw:17
- Flush:17: COTS_90044A123_Black-Oxide Alloy Steel Socket Head Screw:15 ↔ COTS_90044A123_Black-Oxide Alloy Steel Socket Head Screw:16
- Mate:138: COTS_90044A120_Black-Oxide Alloy Steel Socket Head Screw:5 ↔ STRU_009_FrameBracket_90:4
- Mate:139: COTS_90044A123_Black-Oxide Alloy Steel Socket Head Screw:11 ↔ STRU_009_FrameBracket_90:4
- Flush:18: COTS_90044A123_Black-Oxide Alloy Steel Socket Head Screw:10 ↔ COTS_90044A123_Black-Oxide Alloy Steel Socket Head Screw:11
- Flush:19: COTS_90044A123_Black-Oxide Alloy Steel Socket Head Screw:11 ↔ COTS_90044A123_Black-Oxide Alloy Steel Socket Head Screw:13
- Flush:20: COTS_90044A123_Black-Oxide Alloy Steel Socket Head Screw:11 ↔ COTS_90044A123_Black-Oxide Alloy Steel Socket Head Screw:12
- Mate:140: STRU_003_BilletPole_28in_Angled:2 ↔ COTS_90044A120_Black-Oxide Alloy Steel Socket Head Screw:3
- Mate:141: COTS_90044A123_Black-Oxide Alloy Steel Socket Head Screw:2 ↔ STRU_009_FrameBracket_90:1
- Mate:142: COTS_90044A120_Black-Oxide Alloy Steel Socket Head Screw:1 ↔ STRU_009_FrameBracket_90:1
- Flush:21: COTS_90044A123_Black-Oxide Alloy Steel Socket Head Screw:2 ↔ COTS_90044A123_Black-Oxide Alloy Steel Socket Head Screw:4
- Flush:22: COTS_90044A123_Black-Oxide Alloy Steel Socket Head Screw:3 ↔ COTS_90044A123_Black-Oxide Alloy Steel Socket Head Screw:4
- Flush:23: COTS_90044A123_Black-Oxide Alloy Steel Socket Head Screw:3 ↔ COTS_90044A123_Black-Oxide Alloy Steel Socket Head Screw:5
- Mate:145: STRU_002_BilletPole_20.56in_Angled:2 ↔ COTS_95615A120_Medium-Strength Steel Nylon-Insert Locknut:7
- Mate:146: STRU_002_BilletPole_20.56in_Angled:2 ↔ COTS_95615A120_Medium-Strength Steel Nylon-Insert Locknut:8
- Mate:147: STRU_002_BilletPole_20.56in_Angled:1 ↔ COTS_95615A120_Medium-Strength Steel Nylon-Insert Locknut:13
- Mate:148: STRU_002_BilletPole_20.56in_Angled:1 ↔ COTS_95615A120_Medium-Strength Steel Nylon-Insert Locknut:14
- Mate:149: STRU_003_BilletPole_28in_Angled_Unique:1 ↔ COTS_95615A120_Medium-Strength Steel Nylon-Insert Locknut:15
- Mate:150: STRU_003_BilletPole_28in_Angled_Unique:1 ↔ COTS_95615A120_Medium-Strength Steel Nylon-Insert Locknut:16
- Mate:151: STRU_003_BilletPole_28in_Angled_Unique:1 ↔ COTS_95615A120_Medium-Strength Steel Nylon-Insert Locknut:6
- Mate:152: STRU_003_BilletPole_28in_Angled_Unique:1 ↔ COTS_95615A120_Medium-Strength Steel Nylon-Insert Locknut:5
- Mate:153: STRU_003_BilletPole_28in_Angled:2 ↔ COTS_95615A120_Medium-Strength Steel Nylon-Insert Locknut:2
- Mate:154: STRU_003_BilletPole_28in_Angled:2 ↔ COTS_95615A120_Medium-Strength Steel Nylon-Insert Locknut:1
- Mate:155: STRU_003_BilletPole_28in_Angled:2 ↔ COTS_95615A120_Medium-Strength Steel Nylon-Insert Locknut:9
- Mate:156: STRU_003_BilletPole_28in_Angled:2 ↔ COTS_95615A120_Medium-Strength Steel Nylon-Insert Locknut:10
- Mate:157: STRU_003_BilletPole_28in_Angled:2 ↔ STRU_001_BilletBlock:10
- Mate:158: STRU_003_BilletPole_28in_Angled:2 ↔ COTS_90044A120_Black-Oxide Alloy Steel Socket Head Screw:3
- Mate:159: STRU_003_BilletPole_28in_Angled_Unique:1 ↔ STRU_001_BilletBlock:11
- Mate:160: STRU_003_BilletPole_28in_Angled_Unique:1 ↔ STRU_001_BilletBlock:12
- Mate:161: STRU_003_BilletPole_28in_Angled:2 ↔ STRU_001_BilletBlock:13
- Mate:162: STRU_001_BilletBlock:13 ↔ COTS_90044A120_Black-Oxide Alloy Steel Socket Head Screw:10
- Mate:163: STRU_003_BilletPole_28in_Angled:2 ↔ STRU_001_BilletBlock:13
- Mate:164: STRU_003_BilletPole_28in_Angled_Unique:1 ↔ STRU_001_BilletBlock:12
- Mate:165: STRU_003_BilletPole_28in_Angled_Unique:1 ↔ STRU_001_BilletBlock:11
- Mate:168: STRU_003_BilletPole_28in_Angled:2 ↔ COTS_90044A120_Black-Oxide Alloy Steel Socket Head Screw:10
- Mate:171: STRU_001_BilletBlock:11 ↔ STRU_007_BilletPole_11in:3
- Mate:172: STRU_001_BilletBlock:10 ↔ STRU_007_BilletPole_11in:3
- Mate:173: STRU_003_BilletPole_28in_Angled:2 ↔ STRU_007_BilletPole_11in:3
- Mate:174: STRU_001_BilletBlock:12 ↔ STRU_007_BilletPole_11in:4
- Mate:175: STRU_001_BilletBlock:13 ↔ STRU_007_BilletPole_11in:4
- Flush:24: STRU_003_BilletPole_28in_Angled:2 ↔ STRU_007_BilletPole_11in:4
- Mate:176: STRU_003_BilletPole_28in_Angled:2 ↔ STRU_007_BilletPole_11in:4
- Mate:177: STRU_009_FrameBracket_90:1 ↔ STRU_006_BilletPole_SwerveOffset:1
- Mate:178: STRU_003_BilletPole_28in_Angled:2 ↔ STRU_006_BilletPole_SwerveOffset:1
- Mate:179: STRU_004_DoubleBillet_90_2.25in:4 ↔ STRU_006_BilletPole_SwerveOffset:1
- Mate:180: STRU_001_BilletBlock:4 ↔ STRU_006_BilletPole_SwerveOffset:1
- Mate:181: STRU_001_BilletBlock:4 ↔ STRU_006_BilletPole_SwerveOffset:1
- Flush:25: STRU_001_BilletBlock:4 ↔ STRU_006_BilletPole_SwerveOffset:1
- Mate:182: STRU_003_BilletPole_28in_Angled:2 ↔ STRU_006_BilletPole_SwerveOffset:2
- Mate:183: STRU_009_FrameBracket_90:4 ↔ STRU_006_BilletPole_SwerveOffset:2
- Mate:184: STRU_004_DoubleBillet_90_2.25in:3 ↔ STRU_006_BilletPole_SwerveOffset:2
- Mate:185: STRU_001_BilletBlock:3 ↔ STRU_006_BilletPole_SwerveOffset:2
- Mate:186: STRU_001_BilletBlock:3 ↔ STRU_006_BilletPole_SwerveOffset:2
- Flush:26: STRU_001_BilletBlock:3 ↔ STRU_006_BilletPole_SwerveOffset:2
- Mate:187: COTS_90044A123_Black-Oxide Alloy Steel Socket Head Screw:11 ↔ STRU_009_FrameBracket_90:4
- Mate:188: COTS_90044A123_Black-Oxide Alloy Steel Socket Head Screw:10 ↔ STRU_009_FrameBracket_90:4
- Mate:189: COTS_95615A120_Medium-Strength Steel Nylon-Insert Locknut:11 ↔ STRU_006_BilletPole_SwerveOffset:2
- Mate:190: COTS_95615A120_Medium-Strength Steel Nylon-Insert Locknut:12 ↔ STRU_006_BilletPole_SwerveOffset:2
- Mate:191: COTS_90044A123_Black-Oxide Alloy Steel Socket Head Screw:3 ↔ STRU_009_FrameBracket_90:1
- Mate:192: COTS_90044A123_Black-Oxide Alloy Steel Socket Head Screw:5 ↔ STRU_009_FrameBracket_90:1
- Mate:193: COTS_90044A120_Black-Oxide Alloy Steel Socket Head Screw:1 ↔ STRU_009_FrameBracket_90:1
- Mate:194: COTS_95615A120_Medium-Strength Steel Nylon-Insert Locknut:3 ↔ STRU_006_BilletPole_SwerveOffset:1
- Mate:195: COTS_95615A120_Medium-Strength Steel Nylon-Insert Locknut:4 ↔ STRU_006_BilletPole_SwerveOffset:1
- Flush:27: STRU_003_BilletPole_28in_Angled_Unique:1 ↔ STRU_007_BilletPole_11in:3
- Mate:200: STRU_002_BilletPole_20.56in_Angled:2 ↔ STRU_011_BilletWedge:1
- Mate:201: STRU_002_BilletPole_20.56in_Angled:2 ↔ STRU_011_BilletWedge:1
- Mate:203: STRU_003_BilletPole_28in_Angled_Unique:1 ↔ STRU_011_BilletWedge:3
- Mate:205: STRU_003_BilletPole_28in_Angled_Unique:1 ↔ STRU_011_BilletWedge:3
- Mate:206: STRU_003_BilletPole_28in_Angled_Unique:1 ↔ STRU_011_BilletWedge:4
- Mate:208: STRU_003_BilletPole_28in_Angled_Unique:1 ↔ STRU_011_BilletWedge:4
- Mate:209: STRU_002_BilletPole_20.56in_Angled:1 ↔ STRU_011_BilletWedge:5
- Mate:211: STRU_002_BilletPole_20.56in_Angled:1 ↔ STRU_011_BilletWedge:5
- Mate:212: STRU_002_BilletPole_20.56in_Angled:1 ↔ COTS_90044A119_Black-Oxide Alloy Steel Socket Head Screw:1
- Mate:213: STRU_002_BilletPole_20.56in_Angled:1 ↔ COTS_90044A119_Black-Oxide Alloy Steel Socket Head Screw:1
- Mate:214: STRU_003_BilletPole_28in_Angled_Unique:1 ↔ COTS_90044A119_Black-Oxide Alloy Steel Socket Head Screw:2
- Mate:215: STRU_003_BilletPole_28in_Angled_Unique:1 ↔ COTS_90044A119_Black-Oxide Alloy Steel Socket Head Screw:2
- Mate:216: STRU_003_BilletPole_28in_Angled_Unique:1 ↔ COTS_90044A119_Black-Oxide Alloy Steel Socket Head Screw:3
- Mate:217: STRU_003_BilletPole_28in_Angled_Unique:1 ↔ COTS_90044A119_Black-Oxide Alloy Steel Socket Head Screw:3
- Mate:218: STRU_002_BilletPole_20.56in_Angled:2 ↔ COTS_90044A119_Black-Oxide Alloy Steel Socket Head Screw:4
- Mate:219: STRU_002_BilletPole_20.56in_Angled:2 ↔ COTS_90044A119_Black-Oxide Alloy Steel Socket Head Screw:4
- Flush:28: STRU_003_BilletPole_28in_Angled_Unique:1 ↔ STRU_012_BilletPoleMiddle:6
- Mate:221: STRU_003_BilletPole_28in_Angled_Unique:1 ↔ STRU_012_BilletPoleMiddle:6
- Flush:29: STRU_003_BilletPole_28in_Angled_Unique:1 ↔ STRU_012_BilletPoleMiddle:5
- Mate:223: STRU_003_BilletPole_28in_Angled_Unique:1 ↔ STRU_012_BilletPoleMiddle:5
- Mate:228: STRU_012_BilletPoleMiddle:6 ↔ STRU_001_BilletBlock:14
- Mate:229: STRU_012_BilletPoleMiddle:6 ↔ STRU_001_BilletBlock:14
- Flush:30: STRU_012_BilletPoleMiddle:6 ↔ STRU_001_BilletBlock:14
- Mate:230: STRU_012_BilletPoleMiddle:5 ↔ STRU_001_BilletBlock:15
- Mate:231: STRU_012_BilletPoleMiddle:5 ↔ STRU_001_BilletBlock:15
- Flush:31: STRU_012_BilletPoleMiddle:5 ↔ STRU_001_BilletBlock:15
- Flush:39: STRU_012_BilletPoleMiddle:5 ↔ STRU_013_BilletCrossbar2_Angled:1
- Mate:233: STRU_012_BilletPoleMiddle:5 ↔ STRU_013_BilletCrossbar2_Angled:1
- Mate:234: STRU_012_BilletPoleMiddle:5 ↔ STRU_013_BilletCrossbar2_Angled:1
- Flush:43: STRU_012_BilletPoleMiddle:6 ↔ STRU_013_BilletCrossbar2_Angled:3
- Mate:249: STRU_012_BilletPoleMiddle:5 ↔ COTS_90044A120_Black-Oxide Alloy Steel Socket Head Screw:11
- Mate:251: STRU_012_BilletPoleMiddle:6 ↔ COTS_90044A120_Black-Oxide Alloy Steel Socket Head Screw:12
- Mate:252: STRU_013_BilletCrossbar2_Angled:1 ↔ STRU_014_BilletPole_9in_Angled:2
- Mate:253: STRU_012_BilletPoleMiddle:5 ↔ STRU_014_BilletPole_9in_Angled:2
- Flush:48: STRU_012_BilletPoleMiddle:5 ↔ STRU_014_BilletPole_9in_Angled:2
- Mate:254: STRU_013_BilletCrossbar2_Angled:3 ↔ STRU_014_BilletPole_9in_Angled:1
- Mate:255: STRU_012_BilletPoleMiddle:6 ↔ STRU_014_BilletPole_9in_Angled:1
- Flush:49: STRU_012_BilletPoleMiddle:6 ↔ STRU_014_BilletPole_9in_Angled:1
- Mate:257: STRU_015_BilletPole_9in:1 ↔ STRU_001_BilletBlock:19
- Mate:258: STRU_015_BilletPole_9in:1 ↔ STRU_001_BilletBlock:19
- Mate:259: STRU_015_BilletPole_9in:1 ↔ STRU_001_BilletBlock:18
- Mate:260: STRU_015_BilletPole_9in:1 ↔ STRU_001_BilletBlock:18
- Flush:52: STRU_015_BilletPole_9in:1 ↔ STRU_001_BilletBlock:18
- Flush:53: STRU_015_BilletPole_9in:1 ↔ STRU_001_BilletBlock:19
- Mate:261: STRU_003_BilletPole_28in_Angled_Unique:1 ↔ STRU_012_BilletPoleMiddle:6
- Mate:262: STRU_003_BilletPole_28in_Angled_Unique:1 ↔ STRU_012_BilletPoleMiddle:5
- Mate:263: STRU_012_BilletPoleMiddle:6 ↔ COTS_90044A120_Black-Oxide Alloy Steel Socket Head Screw:12
- Mate:264: STRU_012_BilletPoleMiddle:5 ↔ COTS_90044A120_Black-Oxide Alloy Steel Socket Head Screw:11
- Mate:265: STRU_001_BilletBlock:19 ↔ STRU_012_BilletPoleMiddle_Unique:1
- Mate:266: STRU_001_BilletBlock:18 ↔ STRU_012_BilletPoleMiddle_Unique:2
- Mate:267: STRU_001_BilletBlock:16 ↔ STRU_012_BilletPoleMiddle_Unique:1
- Mate:268: STRU_001_BilletBlock:16 ↔ STRU_012_BilletPoleMiddle_Unique:1
- Flush:54: STRU_001_BilletBlock:16 ↔ STRU_012_BilletPoleMiddle_Unique:1
- Mate:269: STRU_001_BilletBlock:17 ↔ STRU_012_BilletPoleMiddle_Unique:2
- Mate:270: STRU_001_BilletBlock:17 ↔ STRU_012_BilletPoleMiddle_Unique:2
- Flush:55: STRU_001_BilletBlock:17 ↔ STRU_012_BilletPoleMiddle_Unique:2
- Mate:271: STRU_001_BilletBlock:18 ↔ STRU_012_BilletPoleMiddle_Unique:2
- Mate:272: STRU_001_BilletBlock:19 ↔ STRU_012_BilletPoleMiddle_Unique:1
- Mate:273: STRU_013_BilletCrossbar2_Angled:1 ↔ STRU_012_BilletPoleMiddle_Unique:2
- Flush:56: STRU_013_BilletCrossbar2_Angled:1 ↔ STRU_012_BilletPoleMiddle_Unique:2
- Flush:57: STRU_013_BilletCrossbar2_Angled:1 ↔ STRU_015_BilletPole_9in:1
- Mate:274: STRU_013_BilletCrossbar2_Angled:3 ↔ STRU_012_BilletPoleMiddle_Unique:1
- Flush:58: STRU_013_BilletCrossbar2_Angled:3 ↔ STRU_012_BilletPoleMiddle_Unique:1
- Mate:275: STRU_001_BilletBlock:18 ↔ COTS_90044A120_Black-Oxide Alloy Steel Socket Head Screw:13
- Mate:276: STRU_001_BilletBlock:19 ↔ COTS_90044A120_Black-Oxide Alloy Steel Socket Head Screw:14
- Mate:277: STRU_012_BilletPoleMiddle_Unique:1 ↔ STRU_016_FrameBracket2_90:1
- Mate:278: STRU_012_BilletPoleMiddle_Unique:1 ↔ STRU_016_FrameBracket2_90:1
- Mate:279: STRU_012_BilletPoleMiddle_Unique:1 ↔ STRU_016_FrameBracket2_90:1
- Mate:280: COTS_90044A120_Black-Oxide Alloy Steel Socket Head Screw:14 ↔ STRU_016_FrameBracket2_90:1
- Mate:281: STRU_012_BilletPoleMiddle_Unique:2 ↔ STRU_016_FrameBracket2_90:2
- Mate:282: STRU_012_BilletPoleMiddle_Unique:2 ↔ STRU_016_FrameBracket2_90:2
- Mate:283: STRU_012_BilletPoleMiddle_Unique:2 ↔ STRU_016_FrameBracket2_90:2
- Mate:284: COTS_90044A120_Black-Oxide Alloy Steel Socket Head Screw:13 ↔ STRU_016_FrameBracket2_90:2
- [Mate]: COTS_90044A123_Black-Oxide Alloy Steel Socket Head Screw:18 ↔ COTS_95615A120_Medium-Strength Steel Nylon-Insert Locknut:17
- Mate:286: STRU_016_FrameBracket2_90:2 ↔ COTS_90044A123_Black-Oxide Alloy Steel Socket Head Screw:18
- Mate:287: STRU_013_BilletCrossbar2_Angled:1 ↔ COTS_95615A120_Medium-Strength Steel Nylon-Insert Locknut:17
- Mate:288: STRU_016_FrameBracket2_90:2 ↔ COTS_90044A123_Black-Oxide Alloy Steel Socket Head Screw:18
- [Mate]: COTS_90044A123_Black-Oxide Alloy Steel Socket Head Screw:19 ↔ COTS_95615A120_Medium-Strength Steel Nylon-Insert Locknut:18
- Mate:290: STRU_016_FrameBracket2_90:2 ↔ COTS_90044A123_Black-Oxide Alloy Steel Socket Head Screw:19
- Mate:291: STRU_014_BilletPole_9in_Angled:2 ↔ COTS_95615A120_Medium-Strength Steel Nylon-Insert Locknut:18
- Mate:292: STRU_016_FrameBracket2_90:2 ↔ COTS_90044A123_Black-Oxide Alloy Steel Socket Head Screw:19
- [Mate]: COTS_90044A123_Black-Oxide Alloy Steel Socket Head Screw:20 ↔ COTS_95615A120_Medium-Strength Steel Nylon-Insert Locknut:19
- Mate:294: STRU_016_FrameBracket2_90:2 ↔ COTS_90044A123_Black-Oxide Alloy Steel Socket Head Screw:20
- Mate:295: STRU_012_BilletPoleMiddle_Unique:2 ↔ COTS_95615A120_Medium-Strength Steel Nylon-Insert Locknut:19
- Mate:296: STRU_016_FrameBracket2_90:2 ↔ COTS_90044A123_Black-Oxide Alloy Steel Socket Head Screw:20
- [Mate]: COTS_90044A123_Black-Oxide Alloy Steel Socket Head Screw:21 ↔ COTS_95615A120_Medium-Strength Steel Nylon-Insert Locknut:20
- Mate:298: STRU_016_FrameBracket2_90:2 ↔ COTS_90044A123_Black-Oxide Alloy Steel Socket Head Screw:21
- Mate:299: STRU_012_BilletPoleMiddle_Unique:2 ↔ COTS_95615A120_Medium-Strength Steel Nylon-Insert Locknut:20
- Mate:300: STRU_016_FrameBracket2_90:2 ↔ COTS_90044A123_Black-Oxide Alloy Steel Socket Head Screw:21
- [Mate]: COTS_90044A123_Black-Oxide Alloy Steel Socket Head Screw:22 ↔ COTS_95615A120_Medium-Strength Steel Nylon-Insert Locknut:21
- Mate:302: STRU_016_FrameBracket2_90:1 ↔ COTS_90044A123_Black-Oxide Alloy Steel Socket Head Screw:22
- Mate:303: STRU_016_FrameBracket2_90:1 ↔ COTS_90044A123_Black-Oxide Alloy Steel Socket Head Screw:22
- Mate:304: STRU_012_BilletPoleMiddle_Unique:1 ↔ COTS_95615A120_Medium-Strength Steel Nylon-Insert Locknut:21
- [Mate]: COTS_90044A123_Black-Oxide Alloy Steel Socket Head Screw:23 ↔ COTS_95615A120_Medium-Strength Steel Nylon-Insert Locknut:22
- Mate:306: STRU_016_FrameBracket2_90:1 ↔ COTS_90044A123_Black-Oxide Alloy Steel Socket Head Screw:23
- Mate:307: STRU_016_FrameBracket2_90:1 ↔ COTS_90044A123_Black-Oxide Alloy Steel Socket Head Screw:23
- Mate:308: STRU_013_BilletCrossbar2_Angled:3 ↔ COTS_95615A120_Medium-Strength Steel Nylon-Insert Locknut:22
- [Mate]: COTS_90044A123_Black-Oxide Alloy Steel Socket Head Screw:24 ↔ COTS_95615A120_Medium-Strength Steel Nylon-Insert Locknut:23
- Mate:310: STRU_016_FrameBracket2_90:1 ↔ COTS_90044A123_Black-Oxide Alloy Steel Socket Head Screw:24
- Mate:311: STRU_014_BilletPole_9in_Angled:1 ↔ COTS_95615A120_Medium-Strength Steel Nylon-Insert Locknut:23
- Mate:312: STRU_016_FrameBracket2_90:1 ↔ COTS_90044A123_Black-Oxide Alloy Steel Socket Head Screw:24
- [Mate]: COTS_90044A123_Black-Oxide Alloy Steel Socket Head Screw:25 ↔ COTS_95615A120_Medium-Strength Steel Nylon-Insert Locknut:24
- Mate:314: STRU_016_FrameBracket2_90:1 ↔ COTS_90044A123_Black-Oxide Alloy Steel Socket Head Screw:25
- Mate:315: STRU_016_FrameBracket2_90:1 ↔ COTS_90044A123_Black-Oxide Alloy Steel Socket Head Screw:25
- Mate:316: STRU_012_BilletPoleMiddle_Unique:1 ↔ COTS_95615A120_Medium-Strength Steel Nylon-Insert Locknut:24
- Mate:317: STRU_014_BilletPole_9in_Angled:1 ↔ STRU_017_AngleBracket_90_Plastic:1
- Mate:318: STRU_012_BilletPoleMiddle:6 ↔ STRU_017_AngleBracket_90_Plastic:1
- Mate:319: STRU_012_BilletPoleMiddle:5 ↔ STRU_017_AngleBracket_90_Plastic:2
- Mate:320: STRU_014_BilletPole_9in_Angled:2 ↔ STRU_017_AngleBracket_90_Plastic:2
- Mate:321: STRU_012_BilletPoleMiddle:5 ↔ STRU_018_AngleBracket_62:3
- Mate:322: STRU_013_BilletCrossbar2_Angled:1 ↔ STRU_018_AngleBracket_62:3
- Mate:323: STRU_013_BilletCrossbar2_Angled:1 ↔ STRU_018_AngleBracket_62:3
- Mate:324: STRU_012_BilletPoleMiddle:6 ↔ STRU_018_AngleBracket_62:4
- Mate:325: STRU_013_BilletCrossbar2_Angled:3 ↔ STRU_018_AngleBracket_62:4
- Mate:326: STRU_013_BilletCrossbar2_Angled:3 ↔ STRU_018_AngleBracket_62:4
- Mate:327: STRU_013_BilletCrossbar2_Angled:1 ↔ STRU_018_AngleBracket_62:1
- Mate:328: STRU_012_BilletPoleMiddle:5 ↔ STRU_018_AngleBracket_62:1
- Mate:329: STRU_013_BilletCrossbar2_Angled:1 ↔ STRU_018_AngleBracket_62:1
- Mate:330: STRU_013_BilletCrossbar2_Angled:3 ↔ STRU_018_AngleBracket_62:2
- Mate:331: STRU_012_BilletPoleMiddle:6 ↔ STRU_018_AngleBracket_62:2
- Mate:332: STRU_013_BilletCrossbar2_Angled:3 ↔ STRU_018_AngleBracket_62:2
- Mate:333: STRU_014_BilletPole_9in_Angled:1 ↔ COTS_91251A539_Black-Oxide Alloy Steel Socket Head Screw (1):4
- Mate:334: STRU_014_BilletPole_9in_Angled:1 ↔ COTS_91251A539_Black-Oxide Alloy Steel Socket Head Screw (1):4
- Mate:335: STRU_014_BilletPole_9in_Angled:1 ↔ COTS_91251A539_Black-Oxide Alloy Steel Socket Head Screw (1):5
- Mate:336: STRU_014_BilletPole_9in_Angled:1 ↔ COTS_91251A539_Black-Oxide Alloy Steel Socket Head Screw (1):5
- Mate:337: STRU_014_BilletPole_9in_Angled:2 ↔ COTS_91251A539_Black-Oxide Alloy Steel Socket Head Screw (1):1
- Mate:338: STRU_014_BilletPole_9in_Angled:2 ↔ COTS_91251A539_Black-Oxide Alloy Steel Socket Head Screw (1):2
- Mate:339: STRU_014_BilletPole_9in_Angled:2 ↔ COTS_91251A539_Black-Oxide Alloy Steel Socket Head Screw (1):2
- Mate:340: STRU_014_BilletPole_9in_Angled:2 ↔ COTS_91251A539_Black-Oxide Alloy Steel Socket Head Screw (1):1
- Mate:359: STRU_018_AngleBracket_62:2 ↔ COTS_90044A124_Black-Oxide Alloy Steel Socket Head Screw:1
- Mate:360: STRU_018_AngleBracket_62:2 ↔ COTS_90044A124_Black-Oxide Alloy Steel Socket Head Screw:3
- Mate:361: STRU_018_AngleBracket_62:2 ↔ COTS_90044A124_Black-Oxide Alloy Steel Socket Head Screw:2
- Mate:362: STRU_018_AngleBracket_62:2 ↔ COTS_90044A124_Black-Oxide Alloy Steel Socket Head Screw:7
- Mate:363: STRU_018_AngleBracket_62:2 ↔ COTS_90044A124_Black-Oxide Alloy Steel Socket Head Screw:8
- Mate:364: STRU_018_AngleBracket_62:2 ↔ COTS_90044A124_Black-Oxide Alloy Steel Socket Head Screw:9
- Mate:371: COTS_95615A120_Medium-Strength Steel Nylon-Insert Locknut:27 ↔ COTS_90044A124_Black-Oxide Alloy Steel Socket Head Screw:1
- Mate:372: COTS_95615A120_Medium-Strength Steel Nylon-Insert Locknut:26 ↔ COTS_90044A124_Black-Oxide Alloy Steel Socket Head Screw:3
- Mate:373: COTS_95615A120_Medium-Strength Steel Nylon-Insert Locknut:25 ↔ COTS_90044A124_Black-Oxide Alloy Steel Socket Head Screw:2
- Mate:374: COTS_95615A120_Medium-Strength Steel Nylon-Insert Locknut:30 ↔ COTS_90044A124_Black-Oxide Alloy Steel Socket Head Screw:7
- Mate:375: COTS_95615A120_Medium-Strength Steel Nylon-Insert Locknut:29 ↔ COTS_90044A124_Black-Oxide Alloy Steel Socket Head Screw:8
- Mate:376: COTS_95615A120_Medium-Strength Steel Nylon-Insert Locknut:28 ↔ COTS_90044A124_Black-Oxide Alloy Steel Socket Head Screw:9
- Mate:377: STRU_018_AngleBracket_62:4 ↔ COTS_90044A124_Black-Oxide Alloy Steel Socket Head Screw:9
- Mate:378: STRU_018_AngleBracket_62:4 ↔ COTS_90044A124_Black-Oxide Alloy Steel Socket Head Screw:2
- Mate:379: STRU_018_AngleBracket_62:4 ↔ COTS_90044A124_Black-Oxide Alloy Steel Socket Head Screw:7
- Mate:380: STRU_018_AngleBracket_62:4 ↔ COTS_90044A124_Black-Oxide Alloy Steel Socket Head Screw:8
- Mate:381: STRU_018_AngleBracket_62:4 ↔ COTS_90044A124_Black-Oxide Alloy Steel Socket Head Screw:3
- Mate:382: STRU_018_AngleBracket_62:4 ↔ COTS_90044A124_Black-Oxide Alloy Steel Socket Head Screw:1
- Mate:383: STRU_018_AngleBracket_62:2 ↔ COTS_95615A120_Medium-Strength Steel Nylon-Insert Locknut:27
- Mate:384: STRU_018_AngleBracket_62:2 ↔ COTS_95615A120_Medium-Strength Steel Nylon-Insert Locknut:26
- Mate:385: STRU_018_AngleBracket_62:2 ↔ COTS_95615A120_Medium-Strength Steel Nylon-Insert Locknut:25
- Mate:386: STRU_018_AngleBracket_62:2 ↔ COTS_95615A120_Medium-Strength Steel Nylon-Insert Locknut:30
- Mate:387: STRU_018_AngleBracket_62:2 ↔ COTS_95615A120_Medium-Strength Steel Nylon-Insert Locknut:29
- Mate:388: STRU_018_AngleBracket_62:2 ↔ COTS_95615A120_Medium-Strength Steel Nylon-Insert Locknut:28
- Mate:389: STRU_012_BilletPoleMiddle:6 ↔ COTS_90044A123_Black-Oxide Alloy Steel Socket Head Screw:28
- Mate:390: STRU_012_BilletPoleMiddle:6 ↔ COTS_90044A123_Black-Oxide Alloy Steel Socket Head Screw:27
- Mate:391: STRU_012_BilletPoleMiddle:5 ↔ COTS_90044A123_Black-Oxide Alloy Steel Socket Head Screw:30
- Mate:392: STRU_012_BilletPoleMiddle:5 ↔ COTS_90044A123_Black-Oxide Alloy Steel Socket Head Screw:29
- Mate:393: STRU_018_AngleBracket_62:1 ↔ COTS_90044A124_Black-Oxide Alloy Steel Socket Head Screw:4